# Autodesk Inventor assembly: EL2-.200
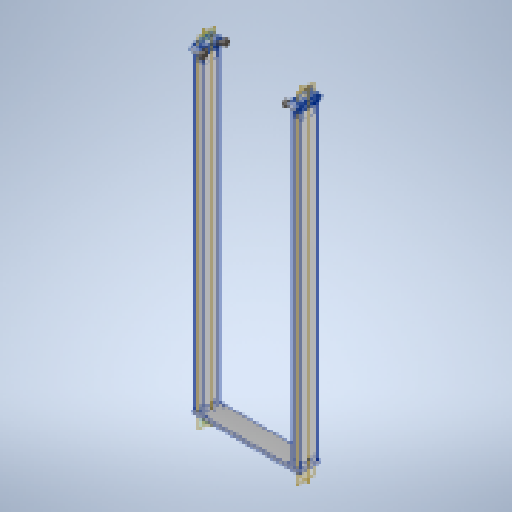
[picture p0: Inventor's stored thumbnail of the model, 512x512]
Saved by Autodesk Inventor 2023.4 (Build 274418000, 418)
## iProperties
Created: 2025-01-11
Part Number: EL2-.200
Document SubType Name: Assembly
Designer: slick
Author: slick
## Documents named in this file (3)
- C:\Users\mavericks\Desktop\2025-ReefScape---CAD\Elevator\EL2\EL2-.200.iam
- C:\Users\mavericks\Desktop\2025-ReefScape---CAD\Elevator\EL2\EL2-003.ipt
- C:\Users\mavericks\Desktop\2025-ReefScape---CAD\Elevator\EL2\EL2-.100.iam
## Components (3 placed, 2 different names)
1. EL2-003:1 — Insert:1, Insert:2, Insert:3, Insert:4
2. EL2-.100:1 [sub-assembly] — Insert:1, Insert:3
3. EL2-.100:2 [sub-assembly] — Insert:2, Insert:4
## Relationships (4: Insert 4)
- Insert:1: EL2-003:1 ↔ EL2-.100:1
- Insert:2: EL2-003:1 ↔ EL2-.100:2
- Insert:3: EL2-003:1 ↔ EL2-.100:1
- Insert:4: EL2-003:1 ↔ EL2-.100:2
